# Autodesk Inventor assembly: Configuration 1
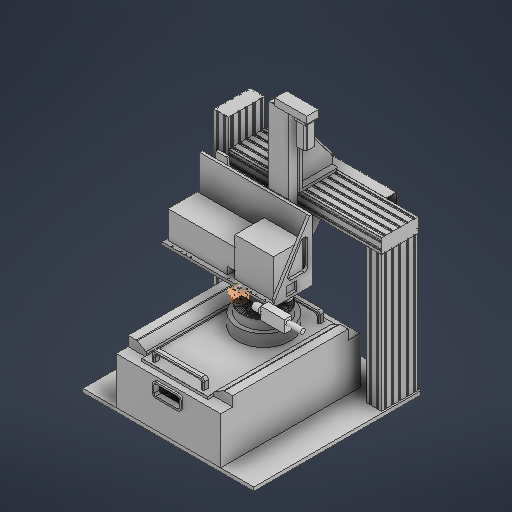
[picture p0: Inventor's stored thumbnail of the model, 512x512]
Saved by Autodesk Inventor 2025 (Build 290162000, 162)
## iProperties
Created: 2024-06-05
Part Number: Configuration 1
Document SubType Name: Assembly
Designer: AdminForWorker
Title: Printer Assembly v13
Author: AdminForWorker
## Documents named in this file (9)
- C:\Users\mayhe\OneDrive\Documents\GitHub\In-situ-monitoring-of-powder-bed-fusion-additive-manufacturing\Laser Bed Fusion Printer CAD\Printer Assembly.iam
- C:\Users\mayhe\OneDrive\Documents\GitHub\In-situ-monitoring-of-powder-bed-fusion-additive-manufacturing\Laser Bed Fusion Printer CAD\Laser w_ silver v4.iam
- C:\Users\mayhe\OneDrive\Documents\GitHub\In-situ-monitoring-of-powder-bed-fusion-additive-manufacturing\Laser Bed Fusion Printer CAD\Printer Body v6.ipt
- C:\Users\mayhe\OneDrive\Documents\GitHub\In-situ-monitoring-of-powder-bed-fusion-additive-manufacturing\Laser Bed Fusion Printer CAD\moving inner chamber piece v1 v2.ipt
- C:\Users\mayhe\OneDrive\Documents\GitHub\In-situ-monitoring-of-powder-bed-fusion-additive-manufacturing\Laser Bed Fusion Printer CAD\Printer Cover v10.iam
- C:\Users\mayhe\OneDrive\Documents\GitHub\In-situ-monitoring-of-powder-bed-fusion-additive-manufacturing\Laser Bed Fusion Printer CAD\Printer Frame.ipt
- C:\Users\mayhe\OneDrive\Documents\GitHub\In-situ-monitoring-of-powder-bed-fusion-additive-manufacturing\system_development\Orichalcum\v0.2\Hardware_design\galvo-scanner\GVS102 Housing.iam
- C:\Users\mayhe\OneDrive\Documents\GitHub\In-situ-monitoring-of-powder-bed-fusion-additive-manufacturing\system_development\Orichalcum\v0.2\Hardware_design\custom-cover\8020-parts\20-2020-200-CL.ipt
- C:\Users\mayhe\OneDrive\Documents\GitHub\In-situ-monitoring-of-powder-bed-fusion-additive-manufacturing\system_development\Orichalcum\v0.2\Hardware_design\laser-vibrometer\Updated Laser Scanner.ipt
## Components (8 placed, 8 different names)
1. Laser w/ silver v4:1 [sub-assembly] — Flush:1, Mate:1, Flush:2
2. Printer Body v6:1
3. moving inner chamber piece v1 v2:1
4. Printer Cover v10:1 [sub-assembly]
5. Part14
6. GVS102 Housing:1 [sub-assembly] — Flush:3, Mate:2
7. 20-2020-200-CL:1 — Flush:1, Mate:1, Flush:2, Flush:3, Mate:2
8. Updated Laser Scanner:2
## Relationships (5: Flush 3, Mate 2)
- Flush:1: Laser w/ silver v4:1 ↔ 20-2020-200-CL:1
- Mate:1: Laser w/ silver v4:1 ↔ 20-2020-200-CL:1
- Flush:2 (10 mm): Laser w/ silver v4:1 ↔ 20-2020-200-CL:1
- Flush:3 (115 mm): GVS102 Housing:1 ↔ 20-2020-200-CL:1
- Mate:2: GVS102 Housing:1 ↔ 20-2020-200-CL:1
